# Autodesk Inventor assembly: DD_KVD_001_AB
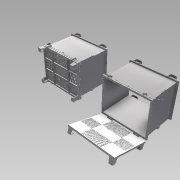
[picture p0: Inventor's stored thumbnail of the model, 180x180]
Saved by Autodesk Inventor 2017.3 (Build 213256000, 256)
## iProperties
Created: 2023-12-15
Part Number: DD_KVD_001_AB
Document SubType Name: Assembly
Designer: Darena
Author: Darena
## Documents named in this file (3)
- D:\2_Darena\1_Soukrome\02_Inventor soukromé\Dílna RAKO3\Záhora\Pivovar KONTEJNER\S výklopným dnem\DD_KVD_001\DD_KVD_001_AB.iam
- D:\2_Darena\1_Soukrome\02_Inventor soukromé\Dílna RAKO3\Záhora\Pivovar KONTEJNER\S výklopným dnem\DD_KVD_001\DD_KVD_001.iam
- D:\2_Darena\1_Soukrome\02_Inventor soukromé\Dílna RAKO3\Záhora\Pivovar KONTEJNER\S výklopným dnem\DD_KVD_001\DD_KVD_001_B.iam
## Components (2 placed, 2 different names)
1. DD_KVD_001:1 [sub-assembly] — Stejný směr:1, Stejný směr:3, Proti sobě:1, Stejný směr:4, Proti sobě:2
2. DD_KVD_001_B:1 [sub-assembly] — Stejný směr:2, Stejný směr:3, Proti sobě:2
## Relationships (6: Flush 4, Mate 2)
- Stejný směr:1 [Flush]: DD_KVD_001:1
- Stejný směr:2 [Flush]: DD_KVD_001_B:1
- Stejný směr:3 [Flush]: DD_KVD_001:1 ↔ DD_KVD_001_B:1
- Proti sobě:1 [Mate]: DD_KVD_001:1
- Stejný směr:4 [Flush] (200 mm): DD_KVD_001:1
- Proti sobě:2 [Mate] (600 mm): DD_KVD_001:1 ↔ DD_KVD_001_B:1
